# Autodesk Inventor assembly: Facing Screw
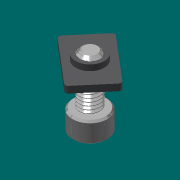
[picture p0: Inventor's stored thumbnail of the model, 180x180]
Saved by Autodesk Inventor 2016 (Build 200138000, 138)
## iProperties
Created: 2015-06-04
Part Number: Facing Screw
Document SubType Name: Assembly
Designer: Sawaiz Syed
Author: Sawaiz Syed
## Documents named in this file (3)
- C:\Users\Sawaiz\Documents\data\projects\cncBlackBox\panels\Facing Screw.iam
- C:\Users\Sawaiz\Documents\data\projects\cncBlackBox\hardware\m5x12.ipt
- C:\Users\Sawaiz\Documents\data\projects\cncBlackBox\hardware\m5TNut.ipt
## Components (2 placed, 2 different names)
1. m5TNut:1 — Mate:2, Mate:3
2. m5x12:1 — Mate:2, Mate:3
## Relationships (2: Mate 2)
- Mate:2 (8.35 mm): m5TNut:1 ↔ m5x12:1
- Mate:3: m5TNut:1 ↔ m5x12:1
